# Autodesk Inventor assembly: SHZA10-30
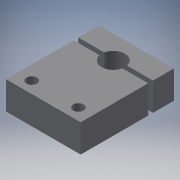
[picture p0: Inventor's stored thumbnail of the model, 180x180]
Saved by Autodesk Inventor 2019 (Build 230136000, 136)
## iProperties
Category: PARTsolutions
Company: MISUMI
Created: 2022-11-15
Part Number: SHZA10-30
Catalog Web Link: www.cadenas.de
Description: SHZB, SHZM, SHZS, SHZA-Shaft Supports - Side Mount - Split
Vendor: MISUMI
Document SubType Name: Assembly
Designer: psAdmin
Manufacturer: MISUMI
Mass: 13.3165 g
Surface Area: 61.6171 cm^2
Volume: 13.3165 cm^3
Density: 1 g/cm^3
Title: SHZA10-30
Author: Cadenas PARTsolutions
Comments: Shaft Supports - Side Mount - Split
PSOL_IDENT_0: {$CADENAS_DATA/23d-libs/misumi/metric/02_shaft_supports/shzb_asmtab.prj},210 {VTYP=3D},{STYP=ASSTAB}
PSOL_IDENT_1: ,{NB=SHZA10-30},{LINA=SHZA10-30},{NN=SHZB, SHZM, SHZS, SHZA},{DATE=30.11.2021 05:41:33},{GEOMDATE=02
PSOL_IDENT_2: .09.2016 03:59:54},{VERSION=},{LINEID=60},{WBVAR=MAT,ST,HS,ALT1,HC},{WBNUMERIC=HS,HC}  {NB=SHZA10-30
PSOL_IDENT_3: },{LINA=SHZA10-30},{KT=DUMMY},{PN=SHZA10-30},{TYPE=SHZA},{MAT=6063},{ST=Clear Anodizing},{AC=Hexagon
PSOL_IDENT_4: Socket Head Cap Screw 2pc (Stainless Steel)},{D=10},{HS=30},{ALT1=-},{HC=0.0},{H=30.0},{L=32},{H1=4
PSOL_IDENT_5: 0.0},{H2=5},{TS=12},{T=12},{TA=12},{L1=20},{DD=4.5},{M=M4 Depth 8},{THMD=4},{THDMIN=3.242},{HCT=},{D
PSOL_IDENT_6: EP=8},{DD2=4.5},{DD1=8},{LL=4.5},{C=2.0},{HM=10.000},{H0=10},{HH=25,'25',30,'30'},{HC1=(25:30/0.1)},
PSOL_IDENT_7: {HCA=0},{HPN=-30},{ALTPN=},{HSALG=25,'25',30,'30'},{HCC1=0},{STA='Clear Anodizing','Clear Anodizing'
PSOL_IDENT_8: },{PPATH=shzb_templ.prj}
NB: SHZA10-30
NN: SHZB, SHZM, SHZS, SHZA
NT: Shaft Supports - Side Mount - Split
NBSYN: $PN.
LINA: SHZA10-30
CATALOG: Misumi
PN: SHZA10-30
MAT: A6063
ST: Clear Anodizing
AC: Hexagon Socket Head Cap Screw 2pc (Stainless Steel)
D: 10
HS: 30
ALT1: w/o HC ( Mounting Height )
HC: 0
H: 30
L: 32
H1: 40
H2: 5
T: 12
L1: 20
DD: 4.5
M: M4 Depth 8
DD2: 4.5
DD1: 8
LL: 4.5
C: 2
SUPPLIER: MISUMI
ARTICLENO: SHZA10-30
BOMINFO: SHZA10-30
CREATOR: CADENAS GmbH
## Documents named in this file (4)
- e:\temp\worker_COMMON_2\temp\tmp_8908_116_3YCrV\format_0\SHZA10-30.iam
- e:\temp\worker_COMMON_2\temp\tmp_8908_116_3YCrV\format_0\SHZA10-30_b.ipt
- e:\temp\worker_COMMON_2\temp\tmp_8908_116_3YCrV\format_0\Slotted head cap screw ISO 4762 - M4x10.ipt
- e:\temp\worker_COMMON_2\temp\tmp_8908_116_3YCrV\format_0\SHZA10-30_p.ipt
## Components (4 placed, 3 different names)
1. SHZA10-30_b:1 — bolt_to_body_Z@1 <-> IP1_Z@2, bolt2_to_body_Z@1 <-> IP1_Z@3, p_to_body_Z@1 <-> p_to_b_Z@4, p_to_body_YZ@1 <-> p_to_b_YZ@4
2. Slotted head cap screw ISO 4762 - M4x10:1 — bolt_to_body_Z@1 <-> IP1_Z@2
3. Slotted head cap screw ISO 4762 - M4x10:2 — bolt2_to_body_Z@1 <-> IP1_Z@3
4. SHZA10-30_p:1 — p_to_body_Z@1 <-> p_to_b_Z@4, p_to_body_YZ@1 <-> p_to_b_YZ@4
## Relationships (4: Mate 3, Angle 1)
- bolt_to_body_Z@1 <-> IP1_Z@2 [Mate]: SHZA10-30_b:1 ↔ Slotted head cap screw ISO 4762 - M4x10:1
- bolt2_to_body_Z@1 <-> IP1_Z@3 [Mate]: SHZA10-30_b:1 ↔ Slotted head cap screw ISO 4762 - M4x10:2
- p_to_body_Z@1 <-> p_to_b_Z@4 [Mate]: SHZA10-30_b:1 ↔ SHZA10-30_p:1
- p_to_body_YZ@1 <-> p_to_b_YZ@4 [Angle] (0 deg): SHZA10-30_b:1 ↔ SHZA10-30_p:1
